# Autodesk Inventor assembly: 8 inch mecanum with toughbox (Right)
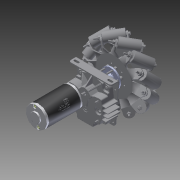
[picture p0: Inventor's stored thumbnail of the model, 180x180]
Saved by Autodesk Inventor 2014 (Build 180170000, 170)
## iProperties
Created: 2015-01-10
Part Number: 8 inch mecanum with toughbox (Right)
Document SubType Name: Assembly
Designer: student
Author: student
## Documents named in this file (6)
- C:\Users\student\Documents\Inventor\2015 Recycle Rush\8 inch mecanum with toughbox (Right).iam
- C:\Users\student\Documents\Inventor\2015 Recycle Rush\am-0077a-500 Key Hub r2_MIR.ipt
- C:\Users\student\Documents\Inventor\2015 Recycle Rush\Derived Toughbox mini_MIR.ipt
- C:\Users\student\Documents\Inventor\Dillon And Justin\Imported Components\MOT_CIM-Motor_217-2000.iam\MOT_CIM-Motor_217-2000.iam.iam
- C:\Users\student\Documents\Inventor\Dillon And Justin\Derived Right Mecanum_MIR.ipt
- MOT_CIM-Motor_217-2000.iam
## Components (4 placed, 4 different names)
1. am-0077a-500 Key Hub r2_MIR:1 — Mate:4, Mate:5, Mate:6, Mate:7
2. Derived Toughbox mini_MIR:1 — Mate:4, Angle:1, Angle:2, Mate:8, Mate:9
3. MOT_CIM-Motor_217-2000.iam:1 [sub-assembly] — Angle:2, Mate:8, Mate:9
4. Derived Right Mecanum_MIR:1 — Mate:5, Mate:6, Mate:7
## Relationships (8: Mate 6, Angle 2)
- Mate:4: am-0077a-500 Key Hub r2_MIR:1 ↔ Derived Toughbox mini_MIR:1
- Angle:1 (0 deg): Derived Toughbox mini_MIR:1
- Mate:5: am-0077a-500 Key Hub r2_MIR:1 ↔ Derived Right Mecanum_MIR:1
- Mate:6: am-0077a-500 Key Hub r2_MIR:1 ↔ Derived Right Mecanum_MIR:1
- Mate:7: am-0077a-500 Key Hub r2_MIR:1 ↔ Derived Right Mecanum_MIR:1
- Angle:2 (180 deg): Derived Toughbox mini_MIR:1 ↔ MOT_CIM-Motor_217-2000.iam:1
- Mate:8: Derived Toughbox mini_MIR:1 ↔ MOT_CIM-Motor_217-2000.iam:1
- Mate:9: Derived Toughbox mini_MIR:1 ↔ MOT_CIM-Motor_217-2000.iam:1
